# Autodesk Inventor assembly: podest duży
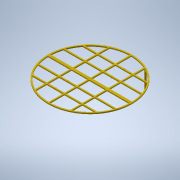
[picture p0: Inventor's stored thumbnail of the model, 180x180]
Saved by Autodesk Inventor 2021 (Build 250183000, 183)
## iProperties
Created: 2024-04-18
Part Number: podest duży
Document SubType Name: Assembly
Designer: Michal
Author: Michal
## Documents named in this file (3)
- C:\Users\Michal\Documents\GitHub\PNW_PhotoBoothFrame_3D\podest duży.iam
- C:\Users\Michal\Documents\GitHub\PNW_PhotoBoothFrame_3D\podest duzy polowka.iam
- C:\Users\Michal\Documents\GitHub\PNW_PhotoBoothFrame_3D\noga podest duzy.iam
## Components (3 placed, 2 different names)
1. podest duzy polowka:1 [sub-assembly] — Flush:1, Flush:2, Mate:1, Mate:2, Flush:3, Mate:3
2. podest duzy polowka:2 [sub-assembly] — Mate:2, Flush:3, Mate:3, Mate:4, Mate:5
3. noga podest duzy:1 [sub-assembly] — Mate:4, Mate:5
## Relationships (8: Mate 5, Flush 3)
- Flush:1: podest duzy polowka:1
- Flush:2: podest duzy polowka:1
- Mate:1: podest duzy polowka:1
- Mate:2: podest duzy polowka:1 ↔ podest duzy polowka:2
- Flush:3: podest duzy polowka:1 ↔ podest duzy polowka:2
- Mate:3: podest duzy polowka:1 ↔ podest duzy polowka:2
- Mate:4: podest duzy polowka:2 ↔ noga podest duzy:1
- Mate:5: podest duzy polowka:2 ↔ noga podest duzy:1
